# Autodesk Inventor assembly: RobotV3
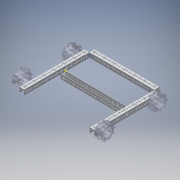
[picture p0: Inventor's stored thumbnail of the model, 180x180]
Saved by Autodesk Inventor 2017 (Build 210142000, 142)
## iProperties
Created: 2017-10-08
Part Number: RobotV3
Document SubType Name: Assembly
Designer: Kenneth
Author: Kenneth
## Documents named in this file (5)
- C:\Workspaces\CAD\RobotV3.iam
- C:\Workspaces\CAD\Spectrum-CAD-Library\FTC\FTC Tetrix KOP\Channel 416mm.ipt
- C:\Workspaces\CAD\Spectrum-CAD-Library\FTC\FTC Tetrix KOP\Bracket L-angle.ipt
- C:\Workspaces\CAD\Spectrum-CAD-Library\FTC\FTC Tetrix KOP\4HD Mecanum Left am-3026L.ipt
- C:\Workspaces\CAD\Spectrum-CAD-Library\FTC\FTC Tetrix KOP\4HD Mecanum Right am-3026R.ipt
## Components (10 placed, 4 different names)
1. Channel 416mm:1 — Mate:1, Mate:2, Mate:6
2. Channel 416mm:2 — Mate:9, Mate:10, Mate:12, Mate:24
3. Channel 416mm:4 — Mate:3, Mate:4, Mate:5, Mate:7, Mate:8, Mate:11, Mate:25
4. Bracket L-angle:2 — Mate:1, Mate:2, Mate:3, Mate:4, Mate:5, Mate:6
5. Bracket L-angle:3 — Mate:7, Mate:8, Mate:9, Mate:10, Mate:11, Mate:12
6. 4HD Mecanum Left am-3026L:1
7. 4HD Mecanum Right am-3026R:1
8. 4HD Mecanum Left am-3026L:2
9. 4HD Mecanum Right am-3026R:2
10. Channel 416mm:5 — Mate:26, Mate:27
## Relationships (16: Mate 16)
- Mate:1: Channel 416mm:1 ↔ Bracket L-angle:2
- Mate:2: Channel 416mm:1 ↔ Bracket L-angle:2
- Mate:3: Channel 416mm:4 ↔ Bracket L-angle:2
- Mate:4: Channel 416mm:4 ↔ Bracket L-angle:2
- Mate:5: Channel 416mm:4 ↔ Bracket L-angle:2
- Mate:6: Channel 416mm:1 ↔ Bracket L-angle:2
- Mate:7: Channel 416mm:4 ↔ Bracket L-angle:3
- Mate:8: Channel 416mm:4 ↔ Bracket L-angle:3
- Mate:9: Channel 416mm:2 ↔ Bracket L-angle:3
- Mate:10: Channel 416mm:2 ↔ Bracket L-angle:3
- Mate:11: Channel 416mm:4 ↔ Bracket L-angle:3
- Mate:12: Channel 416mm:2 ↔ Bracket L-angle:3
- Mate:24: Channel 416mm:2
- Mate:25: Channel 416mm:4
- Mate:26: Channel 416mm:5
- Mate:27: Channel 416mm:5
